# Autodesk Inventor assembly: Assembly1
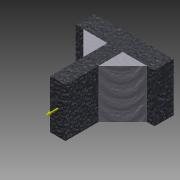
[picture p0: Inventor's stored thumbnail of the model, 180x180]
Saved by Autodesk Inventor 2014 SP2 (Build 180246200, 246)
## iProperties
Created: 2019-07-04
Part Number: Assembly1
Document SubType Name: Weldment
Designer: USER PC
Weld Material: Aluminum 6061, Welded
Author: USER PC
## Documents named in this file (2)
- C:\Users\USER PC\Desktop\United Tractors\New folder\Assembly1.iam
- C:\Users\USER PC\Desktop\United Tractors\New folder\Part1.ipt
## Components (1 placed, 1 different names)
1. Part1:1
## Named parameters: sa_0 = 0, sa_1 = 0, sa_2 = 1.5e+06
note: some values were not read from the file. Shown as the stored number, unit unknown: "sa_0", "sa_1", "sa_2".
